# Autodesk Inventor assembly: ASY PNS680-Filter legs D1000
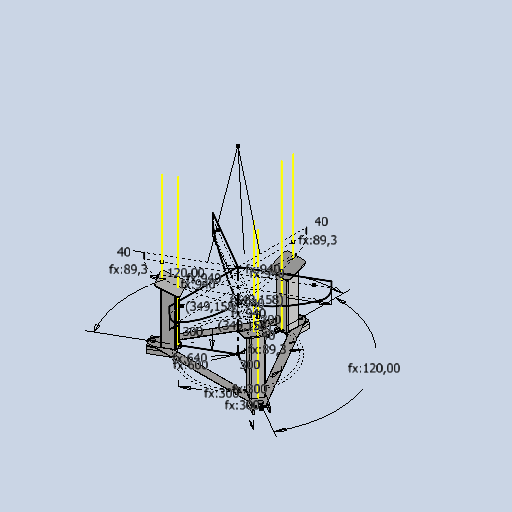
[picture p0: Inventor's stored thumbnail of the model, 512x512]
Saved by Autodesk Inventor 2025 (Build 290162010, 162A)
## iProperties
Created: 2025-02-20
Part Number: ASY PNS680-Filter legs D1000
Document SubType Name: Assembly
Designer: user
Author: user
## Documents named in this file (9)
- C:\Users\admin\Yandex.Disk\home pc\Inventor\PNS2-Panaevsk\Filter D1000\ASY PNS680-Filter legs D1000.iam
- C:\Users\admin\Yandex.Disk\home pc\Inventor\PNS2-Panaevsk\Filter D1000\PNS-681 Leg tube.ipt
- C:\Users\admin\Yandex.Disk\home pc\Inventor\PNS2-Panaevsk\Filter D1000\PNS-689 leg sketch.ipt
- C:\Users\admin\Yandex.Disk\home pc\Inventor\PNS2-Panaevsk\Filter D1000\PNS-682 leg plate for filter.ipt
- C:\Users\admin\Yandex.Disk\home pc\Inventor\PNS2-Panaevsk\Filter D1000\PNS-683 leg floor plate.ipt
- C:\Users\admin\Yandex.Disk\home pc\Inventor\PNS2-Panaevsk\Filter D1200\PNS-785 leg floor channel.ipt
- C:\Users\admin\Yandex.Disk\home pc\Inventor\PNS2-Panaevsk\CC\en-US\DIN EN ISO 8673\DIN EN ISO 8673 - M16 x 1.5.ipt
- C:\Users\admin\Yandex.Disk\home pc\Inventor\PNS2-Panaevsk\CC\en-US\ISO 4017(1)\ISO 4017 - M16 x 40 - ISO.ipt
- C:\Users\admin\Yandex.Disk\home pc\Inventor\PNS2-Panaevsk\Filter D1000\PNS-689 leg floor pattern.ipt
## Components (20 placed, 8 different names)
1. PNS-681 Leg tube.ipt:1 — Mate:2, Mate:8, Tangent:2, Rigid:2, Rigid:5
2. PNS-681 Leg tube.ipt:2 — Mate:4, Mate:7, Tangent:3, Rigid:1, Rigid:4
3. PNS-681 Leg tube.ipt:3 — Mate:3, Mate:6, Tangent:1, Rigid:3, Rigid:6
4. PNS-689 leg sketch.ipt:1 — Mate:6, Tangent:1, Mate:7, Mate:8, Tangent:2, Tangent:3
5. PNS-682 leg plate for filter.ipt:1 — Rigid:1
6. PNS-682 leg plate for filter.ipt:2 — Rigid:2
7. PNS-682 leg plate for filter.ipt:3 — Rigid:3
8. PNS-683 leg floor plate.ipt:1 — Rigid:4, Rigid:10, Rigid:12, Rotational:4
9. PNS-683 leg floor plate.ipt:2 — Rigid:5, Rigid:7, Rigid:8
10. PNS-683 leg floor plate.ipt:3 — Rigid:6, Rigid:9, Rigid:11
11. PNS-785 leg floor channel:1 — Rigid:10
12. DIN EN ISO 8673 M16 x 1.5:1
13. ISO 4017 M16 x 40:1 — Rigid:11
14. PNS-785 leg floor channel:2 — Rigid:9
15. DIN EN ISO 8673 M16 x 1.5:2
16. ISO 4017 M16 x 40:2 — Rigid:12
17. PNS-785 leg floor channel:3 — Rigid:7
18. DIN EN ISO 8673 M16 x 1.5:3
19. ISO 4017 M16 x 40:3 — Rigid:8
20. PNS-689 leg floor pattern:1 — Rotational:4
## Relationships (25: WeldJoint 12, Mate 6, RevoluteJoint 4, Tangent 3)
- Mate:2: PNS-681 Leg tube.ipt:1
- Mate:3: PNS-681 Leg tube.ipt:3
- Mate:4: PNS-681 Leg tube.ipt:2
- Mate:6: PNS-681 Leg tube.ipt:3 ↔ PNS-689 leg sketch.ipt:1
- Tangent:1: PNS-681 Leg tube.ipt:3 ↔ PNS-689 leg sketch.ipt:1
- Mate:7: PNS-681 Leg tube.ipt:2 ↔ PNS-689 leg sketch.ipt:1
- Mate:8: PNS-681 Leg tube.ipt:1 ↔ PNS-689 leg sketch.ipt:1
- Tangent:2: PNS-681 Leg tube.ipt:1 ↔ PNS-689 leg sketch.ipt:1
- Tangent:3: PNS-681 Leg tube.ipt:2 ↔ PNS-689 leg sketch.ipt:1
- Rigid:1 [WeldJoint]: PNS-681 Leg tube.ipt:2 ↔ PNS-682 leg plate for filter.ipt:1
- Rigid:2 [WeldJoint]: PNS-681 Leg tube.ipt:1 ↔ PNS-682 leg plate for filter.ipt:2
- Rigid:3 [WeldJoint]: PNS-681 Leg tube.ipt:3 ↔ PNS-682 leg plate for filter.ipt:3
- Rigid:4 [WeldJoint]: PNS-681 Leg tube.ipt:2 ↔ PNS-683 leg floor plate.ipt:1
- Rigid:5 [WeldJoint]: PNS-681 Leg tube.ipt:1 ↔ PNS-683 leg floor plate.ipt:2
- Rigid:6 [WeldJoint]: PNS-681 Leg tube.ipt:3 ↔ PNS-683 leg floor plate.ipt:3
- [RevoluteJoint]: PNS-785 leg floor channel:1 ↔ DIN EN ISO 8673 M16 x 1.5:1
- [RevoluteJoint]: PNS-785 leg floor channel:2 ↔ DIN EN ISO 8673 M16 x 1.5:2
- [RevoluteJoint]: PNS-785 leg floor channel:3 ↔ DIN EN ISO 8673 M16 x 1.5:3
- Rigid:7 [WeldJoint]: PNS-683 leg floor plate.ipt:2 ↔ PNS-785 leg floor channel:3
- Rigid:8 [WeldJoint]: PNS-683 leg floor plate.ipt:2 ↔ ISO 4017 M16 x 40:3
- Rigid:9 [WeldJoint]: PNS-683 leg floor plate.ipt:3 ↔ PNS-785 leg floor channel:2
- Rigid:10 [WeldJoint]: PNS-683 leg floor plate.ipt:1 ↔ PNS-785 leg floor channel:1
- Rigid:11 [WeldJoint]: PNS-683 leg floor plate.ipt:3 ↔ ISO 4017 M16 x 40:1
- Rigid:12 [WeldJoint]: PNS-683 leg floor plate.ipt:1 ↔ ISO 4017 M16 x 40:2
- Rotational:4 [RevoluteJoint]: PNS-683 leg floor plate.ipt:1 ↔ PNS-689 leg floor pattern:1
## Named parameters: d22_d30 = 0 mm, d23_d31 = 0 deg, d24_d30 = 0 mm, d25_d31 = 120 deg
